# Autodesk Inventor assembly: reducer_1
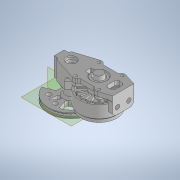
[picture p0: Inventor's stored thumbnail of the model, 180x180]
Saved by Autodesk Inventor 2020 (Build 240168000, 168)
## iProperties
Created: 2021-03-10
Part Number: reducer_1
Document SubType Name: Assembly
Designer: Shuang Peng
Author: Shuang Peng
## Documents named in this file (5)
- D:\projects-3\biped_tiny\hardware\sim_mod\reducer_1.iam
- D:\projects-3\biped_tiny\hardware\mot_holder_1.ipt
- D:\projects-3\biped_tiny\hardware\mot_27_ass.iam
- D:\projects-3\biped_tiny\hardware\tendon_wh_1.ipt
- D:\projects-3\biped_tiny\hardware\tendon_wh_3.ipt
## Components (4 placed, 4 different names)
1. mot_holder_1:1 — Flush:1, Mate:1, Insert:1, Insert:2, Insert:6, Angle:1
2. mot_27_ass:1 [sub-assembly] — Insert:1, Insert:2, Insert:4, Insert:5
3. tendon_wh_1:1 — Insert:4, Insert:5
4. tendon_wh_3:1 — Insert:6, Angle:1
## Relationships (8: Insert 5, Flush 1, Mate 1, Angle 1)
- Flush:1: mot_holder_1:1
- Mate:1: mot_holder_1:1
- Insert:1: mot_holder_1:1 ↔ mot_27_ass:1
- Insert:2: mot_holder_1:1 ↔ mot_27_ass:1
- Insert:4: mot_27_ass:1 ↔ tendon_wh_1:1
- Insert:5: mot_27_ass:1 ↔ tendon_wh_1:1
- Insert:6: mot_holder_1:1 ↔ tendon_wh_3:1
- Angle:1 (180 deg): mot_holder_1:1 ↔ tendon_wh_3:1
